# Autodesk Inventor assembly: tubeClampFinal
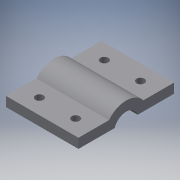
[picture p0: Inventor's stored thumbnail of the model, 180x180]
Saved by Autodesk Inventor 2018 (Build 220112000, 112)
## iProperties
Created: 2017-10-07
Part Number: tubeClampFinal
Document SubType Name: Assembly
Designer: Payal Jindal
Author: Payal Jindal
## Documents named in this file (2)
- C:\Users\Payal Jindal\Documents\Inventor\Mousetrap\tubeClampFinal.iam
- C:\Users\Payal Jindal\Documents\Inventor\Mousetrap\tubeClamp.ipt
## Components (1 placed, 1 different names)
1. tubeClamp:1 — Mate:1, Mate:2
## Relationships (2: Mate 2)
- Mate:1: tubeClamp:1
- Mate:2: tubeClamp:1
